# Autodesk Inventor assembly: bearing_all
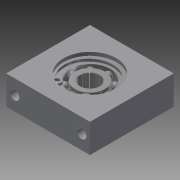
[picture p0: Inventor's stored thumbnail of the model, 180x180]
Saved by Autodesk Inventor 2015 (Build 190159000, 159)
## iProperties
Created: 2015-04-17
Part Number: bearing_all
Document SubType Name: Assembly
Designer: Marcin
Author: Marcin
## Documents named in this file (4)
- C:\Users\Kuba\Dysk Google\synergia\Synergolf\model\GOLF\bearing_all.iam
- C:\Users\Kuba\Dysk Google\synergia\Synergolf\model\GOLF\bearing_frame.ipt
- C:\Users\Kuba\Dysk Google\synergia\Synergolf\model\GOLF\DIN 472 - 22x1.ipt
- C:\Users\Kuba\Dysk Google\synergia\Synergolf\model\GOLF\DIN 630 - 108 - 8 x 22 x 7.ipt
## Components (4 placed, 3 different names)
1. bearing_frame:1 — Zestawiający:1, Zestawiający:2, Równoległy:1, Zestawiający:3, Równoległy:2, Zestawiający:4, Zestawiający:5, Zestawiający:6, Zestawiający:7, Zestawiający:8, Zestawiający:9
2. DIN 472 22x1:1 — Zestawiający:5, Zestawiający:7, Zestawiający:8
3. DIN 472 22x1:2 — Zestawiający:4, Zestawiający:6, Zestawiający:9
4. DIN 630 108 - 8 x 22 x 7:1 — Zestawiający:3, Równoległy:2
## Relationships (11: Mate 9, Flush 2)
- Zestawiający:1 [Mate]: bearing_frame:1
- Zestawiający:2 [Mate]: bearing_frame:1
- Równoległy:1 [Flush]: bearing_frame:1
- Zestawiający:3 [Mate]: bearing_frame:1 ↔ DIN 630 108 - 8 x 22 x 7:1
- Równoległy:2 [Flush]: bearing_frame:1 ↔ DIN 630 108 - 8 x 22 x 7:1
- Zestawiający:4 [Mate]: bearing_frame:1 ↔ DIN 472 22x1:2
- Zestawiający:5 [Mate]: bearing_frame:1 ↔ DIN 472 22x1:1
- Zestawiający:6 [Mate]: bearing_frame:1 ↔ DIN 472 22x1:2
- Zestawiający:7 [Mate]: bearing_frame:1 ↔ DIN 472 22x1:1
- Zestawiający:8 [Mate]: bearing_frame:1 ↔ DIN 472 22x1:1
- Zestawiający:9 [Mate]: bearing_frame:1 ↔ DIN 472 22x1:2
